# Autodesk Inventor assembly: A2017_T2_01
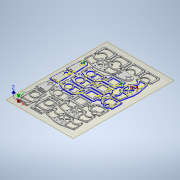
[picture p0: Inventor's stored thumbnail of the model, 180x180]
Saved by Autodesk Inventor 2020 (Build 240168000, 168)
## iProperties
Created: 2021-08-27
Part Number: A2017_T2_01
Document SubType Name: Assembly
Designer: Masato
Author: Masato
## Documents named in this file (9)
- C:\Users\naoki\Documents\Inventor\CitBrains\git_clone\OpenPlatform4_0\CAM\OpenPlatform_ver3_0\cam\A2017_T2_01.iam
- C:\Users\naoki\Documents\Inventor\CitBrains\git_clone\OpenPlatform4_0\CAM\OpenPlatform_ver3_0\cam\Disposable_Board.ipt
- C:\Users\naoki\Documents\Inventor\CitBrains\git_clone\OpenPlatform4_0\CAM\OpenPlatform_ver3_0\UpperBody\Trunk\Trunk_chest_side_frame.ipt
- C:\Users\naoki\Documents\Inventor\CitBrains\git_clone\OpenPlatform4_0\CAM\OpenPlatform_ver3_0\UpperBody\Trunk\Trunk_chest_horizontal_frame.ipt
- C:\Users\naoki\Documents\Inventor\CitBrains\git_clone\OpenPlatform4_0\CAM\OpenPlatform_ver3_0\UpperBody\Arm\Shoulder_side_frame.ipt
- C:\Users\naoki\Documents\Inventor\CitBrains\git_clone\OpenPlatform4_0\CAM\OpenPlatform_ver3_0\LowerBody\Knee\Knee_side_frame.ipt
- C:\Users\naoki\Documents\Inventor\CitBrains\git_clone\OpenPlatform4_0\CAM\OpenPlatform_ver3_0\LowerBody\Ankle\Ankle_back_frame.ipt
- C:\Users\naoki\Documents\Inventor\CitBrains\git_clone\OpenPlatform4_0\CAM\OpenPlatform_ver3_0\LowerBody\Ankle\Ankle_side_frame.ipt
- C:\Users\naoki\Documents\Inventor\CitBrains\git_clone\OpenPlatform4_0\CAM\OpenPlatform_ver3_0\LowerBody\Foot\Foot_back_frame.ipt
## Components (21 placed, 8 different names)
1. Disposable_Board:1 — メイト:2, メイト:1, フラッシュ:1, フラッシュ:2, フラッシュ:3, フラッシュ:4, フラッシュ:6, フラッシュ:7, フラッシュ:9, 角度:1, メイト:31
2. Shoulder_side_frame:1 — メイト:9, フラッシュ:7, 正接:2, 正接:6
3. Knee_side_frame:3 — 正接:7, 正接:8, メイト:30, 角度:1, 正接:9, 正接:10
4. Knee_side_frame:4 — 正接:11, 正接:12
5. Shoulder_side_frame:2 — メイト:31, メイト:32, 正接:10
6. Trunk_chest_horizontal_frame:1 — フラッシュ:3, メイト:4, フラッシュ:4, フラッシュ:10
7. Trunk_chest_horizontal_frame:2 — メイト:6
8. Knee_side_frame:1 — フラッシュ:6, メイト:5, メイト:6
9. Knee_side_frame:2 — メイト:8, 正接:1, 正接:3
10. Trunk_chest_side_frame:1 — メイト:11, メイト:12, 正接:3
11. Trunk_chest_side_frame:2 — 正接:12
12. Ankle_side_frame:1 — メイト:7, メイト:8, 正接:1, 正接:2, メイト:12
13. Ankle_side_frame:2
14. Ankle_side_frame:3 — 正接:11
15. Ankle_side_frame:4 — 正接:8, メイト:32
16. Foot_back_frame:1 — メイト:16, フラッシュ:9, 正接:6
17. Foot_back_frame:3
18. Ankle_back_frame:3 — メイト:29, 正接:7, フラッシュ:10, 正接:9
19. Ankle_back_frame:4
20. Ankle_back_frame:5
21. Ankle_back_frame:6
## Component patterns: (2 elements, first: Trunk_chest_horizontal_frame:1), (2 elements, first: Knee_side_frame:1), (2 elements, first: Trunk_chest_side_frame:1), (4 elements, first: Ankle_side_frame:1), (2 elements, first: Foot_back_frame:1), (4 elements, first: Ankle_back_frame:3)
## Relationships (34: Mate 15, Tangent 10, Flush 8, Angle 1)
- メイト:2 [Mate]: Disposable_Board:1
- メイト:1 [Mate]: Disposable_Board:1
- フラッシュ:1 [Flush]: Disposable_Board:1
- フラッシュ:2 [Flush]: Disposable_Board:1
- フラッシュ:3 [Flush] (2 mm): Disposable_Board:1 ↔ Trunk_chest_horizontal_frame:1
- メイト:4 [Mate]: Trunk_chest_horizontal_frame:1
- フラッシュ:4 [Flush] (2 mm): Disposable_Board:1 ↔ Trunk_chest_horizontal_frame:1
- フラッシュ:6 [Flush] (2 mm): Disposable_Board:1 ↔ Knee_side_frame:1
- メイト:5 [Mate]: Knee_side_frame:1
- メイト:6 [Mate] (2.5 mm): Trunk_chest_horizontal_frame:2 ↔ Knee_side_frame:1
- メイト:7 [Mate]: Ankle_side_frame:1
- メイト:8 [Mate] (5 mm): Knee_side_frame:2 ↔ Ankle_side_frame:1
- 正接:1 [Tangent] (2.5 mm): Knee_side_frame:2 ↔ Ankle_side_frame:1
- メイト:9 [Mate]: Shoulder_side_frame:1
- フラッシュ:7 [Flush] (2 mm): Disposable_Board:1 ↔ Shoulder_side_frame:1
- 正接:2 [Tangent] (2.3 mm): Shoulder_side_frame:1 ↔ Ankle_side_frame:1
- メイト:11 [Mate]: Trunk_chest_side_frame:1
- メイト:12 [Mate] (2.5 mm): Trunk_chest_side_frame:1 ↔ Ankle_side_frame:1
- 正接:3 [Tangent] (2.5 mm): Knee_side_frame:2 ↔ Trunk_chest_side_frame:1
- メイト:16 [Mate]: Foot_back_frame:1
- メイト:29 [Mate]: Ankle_back_frame:3
- フラッシュ:9 [Flush] (2 mm): Disposable_Board:1 ↔ Foot_back_frame:1
- 正接:6 [Tangent] (2.5 mm): Shoulder_side_frame:1 ↔ Foot_back_frame:1
- 正接:7 [Tangent] (2.5 mm): Knee_side_frame:3 ↔ Ankle_back_frame:3
- フラッシュ:10 [Flush]: Trunk_chest_horizontal_frame:1 ↔ Ankle_back_frame:3
- 正接:8 [Tangent] (2.5 mm): Knee_side_frame:3 ↔ Ankle_side_frame:4
- メイト:30 [Mate]: Knee_side_frame:3
- 角度:1 [Angle] (0 deg): Disposable_Board:1 ↔ Knee_side_frame:3
- 正接:9 [Tangent]: Knee_side_frame:3 ↔ Ankle_back_frame:3
- メイト:31 [Mate]: Disposable_Board:1 ↔ Shoulder_side_frame:2
- メイト:32 [Mate] (2.5 mm): Shoulder_side_frame:2 ↔ Ankle_side_frame:4
- 正接:10 [Tangent] (2.5 mm): Knee_side_frame:3 ↔ Shoulder_side_frame:2
- 正接:11 [Tangent] (2.5 mm): Knee_side_frame:4 ↔ Ankle_side_frame:3
- 正接:12 [Tangent] (2.5 mm): Knee_side_frame:4 ↔ Trunk_chest_side_frame:2
